# Autodesk Inventor assembly: PWTR-0044
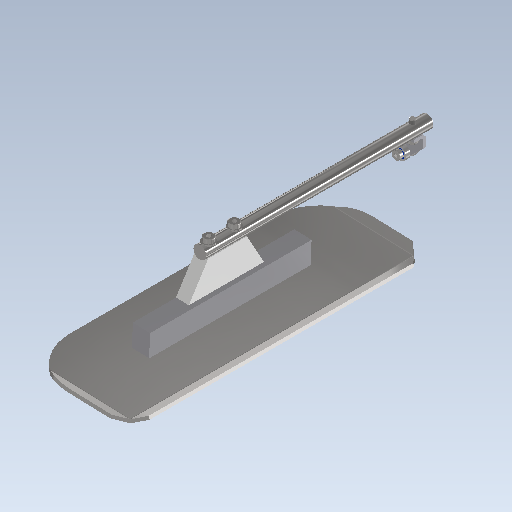
[picture p0: Inventor's stored thumbnail of the model, 512x512]
Saved by Autodesk Inventor 2021.1 (Build 251245010, 245A)
## iProperties
Created: 2020-08-27
Part Number: PWTR-0044
Document SubType Name: Assembly
Designer: alid
Description: Trowel Assembly
Author: alid
## Documents named in this file (12)
- C:\Users\peter\source\repos\InventorDA-FLC\Dataset\FY2021 Power Trowel\PWTR-0044.iam
- C:\Users\peter\source\repos\InventorDA-FLC\Dataset\FY2021 Power Trowel\PWTR-0031.ipt
- C:\Users\peter\source\repos\InventorDA-FLC\Dataset\FY2021 Power Trowel\PWTR-0036.ipt
- C:\Users\peter\source\repos\InventorDA-FLC\Dataset\FY2021 Power Trowel\PWTR-0029.ipt
- C:\Users\peter\source\repos\InventorDA-FLC\Dataset\FY2021 Power Trowel\PWTR-0039.ipt
- C:\Users\peter\source\repos\InventorDA-FLC\Dataset\FY2021 Power Trowel\PWTR-0034.ipt
- C:\Users\peter\source\repos\InventorDA-FLC\Dataset\FY2021 Power Trowel\PWTR-0042.ipt
- C:\Users\peter\source\repos\InventorDA-FLC\Dataset\FY2021 Power Trowel\PWTR-0041.ipt
- C:\Users\peter\source\repos\InventorDA-FLC\Dataset\FY2021 Power Trowel\PWTR-0154.ipt
- C:\Users\peter\source\repos\InventorDA-FLC\Dataset\FY2021 Power Trowel\PWTR-0155.ipt
- C:\Users\peter\source\repos\InventorDA-FLC\Dataset\FY2021 Power Trowel\PWTR-0156.ipt
- C:\Users\peter\source\repos\InventorDA-FLC\Dataset\FY2021 Power Trowel\PWTR-0153.ipt
## Components (14 placed, 11 different names)
1. Trowel Arm — Insert:2, Insert:3
2. PWTR-0036:1
3. PWTR-0029:1
4. PWTR-0039:1
5. PWTR-0034:1
6. PWTR-0029:2
7. DIN 7984 M6 x 16:1
8. DIN 7984 M5 x 20:1
9. PWTR-0155:1 — Insert:4
10. PWTR-0155:2 — Insert:5
11. DIN 128 A6:1 — Insert:2, Insert:4
12. DIN 128 A6:2 — Insert:3, Insert:5
13. TROWEL — Mate:13, Flush:1
14. TROWEL SUPPORT — Mate:13, Flush:1
## Relationships (21: Mate 13, Insert 7, Flush 1)
- [Insert]: PWTR-0036:1 ↔ DIN 7984 M6 x 16:1
- [Mate]: Trowel Arm ↔ PWTR-0039:1
- [Mate]: PWTR-0039:1 ↔ TROWEL SUPPORT
- [Mate]: Trowel Arm ↔ PWTR-0039:1
- Insert:2: Trowel Arm ↔ DIN 128 A6:1
- Insert:3: Trowel Arm ↔ DIN 128 A6:2
- Insert:4: PWTR-0155:1 ↔ DIN 128 A6:1
- Insert:5: PWTR-0155:2 ↔ DIN 128 A6:2
- [Mate]: PWTR-0036:1 ↔ PWTR-0029:1
- [Mate]: PWTR-0155:1 ↔ TROWEL SUPPORT
- [Mate]: PWTR-0155:2 ↔ TROWEL SUPPORT
- [Mate]: Trowel Arm ↔ DIN 7984 M6 x 16:1
- [Mate]: PWTR-0036:1 ↔ PWTR-0029:2
- [Mate]: PWTR-0029:2 ↔ DIN 7984 M5 x 20:1
- [Insert]: PWTR-0034:1 ↔ PWTR-0029:2
- [Mate]: PWTR-0036:1 ↔ DIN 7984 M5 x 20:1
- [Mate]: Trowel Arm ↔ PWTR-0036:1
- [Insert]: PWTR-0029:1 ↔ DIN 7984 M5 x 20:1
- [Mate]: TROWEL ↔ TROWEL SUPPORT
- Mate:13: TROWEL ↔ TROWEL SUPPORT
- Flush:1: TROWEL ↔ TROWEL SUPPORT
## Named parameters: d0_d1 = 0 mm, d1_d3 = 0 mm, d2_d8 = 0 mm, d71_d87 = 0 mm
